# Autodesk Inventor assembly: ABD_Slider_Set
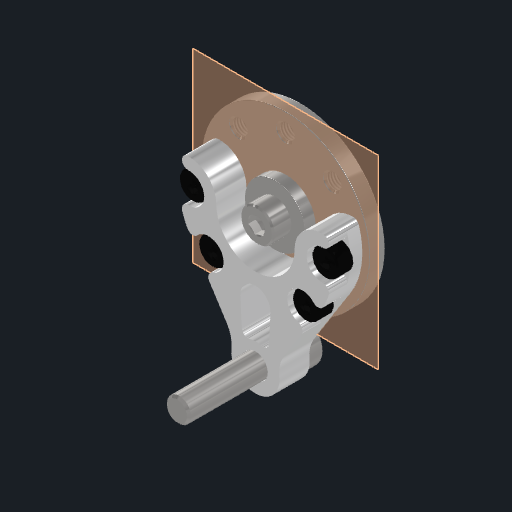
[picture p0: Inventor's stored thumbnail of the model, 512x512]
Saved by Autodesk Inventor 2024.3 (Build 283343000, 343)
## iProperties
Created: 2024-02-15
Part Number: ABD_Slider_Set
Document SubType Name: Assembly
Designer: ASUS
Author: ASUS
## Documents named in this file (6)
- C:\Users\ASUS\Desktop\DK\Anti_Backlash_Structure_OP\v2_Frame\ABD_Slider_Set_v2.iam
- C:\Users\ASUS\Desktop\DK\Anti_Backlash_Structure_OP\ROBOTIS(Inventor 2024 ver.)\HORN\64-106Horn.ipt
- C:\Users\ASUS\Desktop\DK\Anti_Backlash_Structure_OP\v2_Frame\Slider_crank_horn_v2.ipt
- C:\Users\ASUS\Desktop\DK\Anti_Backlash_Structure_OP\v2_Frame\MISUMI\CSH-STN-M3-10.ipt
- C:\Users\ASUS\Desktop\DK\Anti_Backlash_Structure_OP\v1_Frame\MISUMI\CSH-ST-M2_5-4.ipt
- C:\Users\ASUS\Desktop\DK\Anti_Backlash_Structure_OP\v2_Frame\MISUMI\CSHBTT-ST-M4-18.ipt
## Components (8 placed, 5 different names)
1. 64-106Horn:1 — 삽입:3, 삽입:6, 메이트:1
2. Slider_crank_horn_v2:1 — 삽입:6, 메이트:1, 삽입:7, 삽입:8, 삽입:9, 삽입:10, 삽입:11
3. CSH-STN-M3-10:1 — 삽입:3
4. CSH-ST-M2_5-4:1 — 삽입:8
5. CSHBTT-ST-M4-18:1 — 삽입:7
6. CSH-ST-M2_5-4:2 — 삽입:10
7. CSH-ST-M2_5-4:3 — 삽입:11
8. CSH-ST-M2_5-4:5 — 삽입:9
## Relationships (8: Insert 7, Mate 1)
- 삽입:3 [Insert]: 64-106Horn:1 ↔ CSH-STN-M3-10:1
- 삽입:6 [Insert]: 64-106Horn:1 ↔ Slider_crank_horn_v2:1
- 메이트:1 [Mate]: 64-106Horn:1 ↔ Slider_crank_horn_v2:1
- 삽입:7 [Insert]: Slider_crank_horn_v2:1 ↔ CSHBTT-ST-M4-18:1
- 삽입:8 [Insert]: Slider_crank_horn_v2:1 ↔ CSH-ST-M2_5-4:1
- 삽입:9 [Insert]: Slider_crank_horn_v2:1 ↔ CSH-ST-M2_5-4:5
- 삽입:10 [Insert]: Slider_crank_horn_v2:1 ↔ CSH-ST-M2_5-4:2
- 삽입:11 [Insert]: Slider_crank_horn_v2:1 ↔ CSH-ST-M2_5-4:3
